# Autodesk Inventor assembly: leg_press_assembly
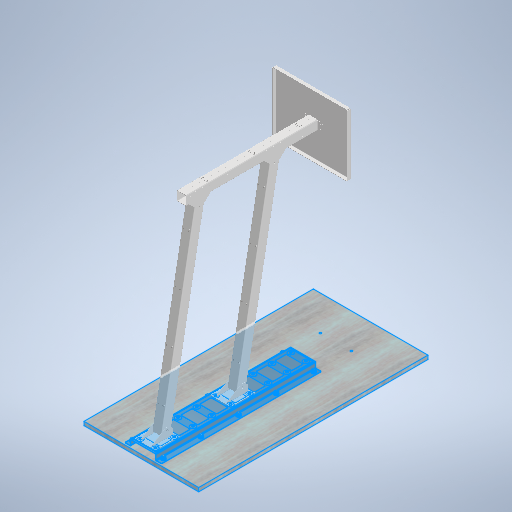
[picture p0: Inventor's stored thumbnail of the model, 512x512]
Saved by Autodesk Inventor 2025.2 (Build 292293000, 293)
## iProperties
Created: 2025-03-24
Part Number: leg_press_assembly
Document SubType Name: Assembly
Designer: Caspe
Author: Caspe
## Documents named in this file (8)
- C:\Users\Caspe\Documents\Semester 8\Project\Anomaly_Detection\Mechanical_Project\Inventor_project\leg_press_assembly.iam
- C:\Users\Caspe\Documents\Semester 8\Project\Anomaly_Detection\Mechanical_Project\Inventor_project\IMS-00-100.iam
- C:\Users\Caspe\Documents\Semester 8\Project\Anomaly_Detection\Mechanical_Project\Inventor_project\bottom_hinge.iam
- C:\Users\Caspe\Documents\Semester 8\Project\Anomaly_Detection\Mechanical_Project\Inventor_project\A1.iam
- C:\Users\Caspe\Documents\Semester 8\Project\Anomaly_Detection\Mechanical_Project\Inventor_project\B_beam.iam
- C:\Users\Caspe\Documents\Semester 8\Project\Anomaly_Detection\Mechanical_Project\Inventor_project\A_B_hinge.ipt
- C:\Users\Caspe\Documents\Semester 8\Project\Anomaly_Detection\Mechanical_Project\Inventor_project\C_plate.ipt
- C:\Users\Caspe\Documents\Semester 8\Project\Anomaly_Detection\Mechanical_Project\Inventor_project\Leg_press_parameters.xlsx
## Components (11 placed, 6 different names)
1. IMS-00-100:1 [sub-assembly] — Insert:1, Insert:2, Insert:3, Insert:4
2. bottom_hinge:1 [sub-assembly] — Insert:1, Insert:2, Mate:1, Mate:2
3. A1:1 [sub-assembly] — Mate:1, Mate:2, Insert:5, Insert:6
4. bottom_hinge:2 [sub-assembly] — Insert:3, Insert:4, Mate:3, Mate:4
5. A1:2 [sub-assembly] — Mate:3, Mate:4, Insert:10, Insert:13
6. B_beam:1 [sub-assembly] — Insert:7, Insert:8, Insert:9, Insert:11, Insert:12, Insert:14, Insert:15, Insert:16, Insert:17
7. A_B_hinge:1 — Insert:5, Insert:7, Insert:8
8. A_B_hinge:2 — Insert:6, Insert:9
9. A_B_hinge:3 — Insert:13, Insert:14, Insert:15
10. A_B_hinge:4 — Insert:10, Insert:11, Insert:12
11. C_plate:1 — Insert:16, Insert:17
## Relationships (21: Insert 17, Mate 4)
- Insert:1: IMS-00-100:1 ↔ bottom_hinge:1
- Insert:2: IMS-00-100:1 ↔ bottom_hinge:1
- Mate:1: bottom_hinge:1 ↔ A1:1
- Mate:2 (3 mm): bottom_hinge:1 ↔ A1:1
- Insert:3: IMS-00-100:1 ↔ bottom_hinge:2
- Insert:4: IMS-00-100:1 ↔ bottom_hinge:2
- Mate:3: bottom_hinge:2 ↔ A1:2
- Mate:4 (3 mm): bottom_hinge:2 ↔ A1:2
- Insert:5 (2 mm): A1:1 ↔ A_B_hinge:1
- Insert:6 (2 mm): A1:1 ↔ A_B_hinge:2
- Insert:7 (2 mm): B_beam:1 ↔ A_B_hinge:1
- Insert:8 (2 mm): B_beam:1 ↔ A_B_hinge:1
- Insert:9 (2 mm): B_beam:1 ↔ A_B_hinge:2
- Insert:10 (2 mm): A1:2 ↔ A_B_hinge:4
- Insert:11 (2 mm): B_beam:1 ↔ A_B_hinge:4
- Insert:12 (2 mm): B_beam:1 ↔ A_B_hinge:4
- Insert:13 (2 mm): A1:2 ↔ A_B_hinge:3
- Insert:14 (2 mm): B_beam:1 ↔ A_B_hinge:3
- Insert:15 (2 mm): B_beam:1 ↔ A_B_hinge:3
- Insert:16: B_beam:1 ↔ C_plate:1
- Insert:17: B_beam:1 ↔ C_plate:1
## Named parameters: A_length = 1000 mm, A_width = 50 mm, A_bend = 20 mm, A_connection_width = 40 mm, A_displacement = 500 mm, A_hole_height = 10 mm, A_hole_length = 40 mm, A_joint_diameter = 10 mm, A_height = 50 mm, A_joint_tolerance = 3 mm, l___________ = 0 mm, B_length = 700 mm, B_width = 50 mm, B_bend = 20 mm, B_connection_width = 40 mm, B_hole_height = 10 mm, B_hole_length = 40 mm, l__________ = 0 mm, C_length = 400 mm, C_width = 20 mm, C_height = 330 mm, l_________ = 0 mm, rivet_diameter = 4 mm, rivet_displacement = 250 mm, plate_thickness = 2 mm, l________ = 0 mm, B_hinge_holes_spacing = 50 mm, B_height = 50 mm, A_B_spacing = 2 mm
